# Autodesk Inventor assembly: CajaElectronica
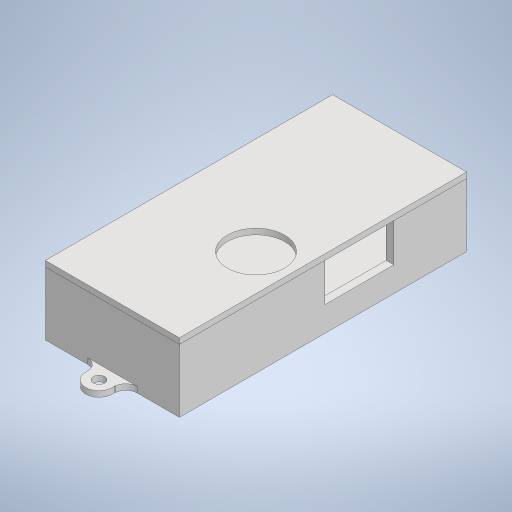
[picture p0: Inventor's stored thumbnail of the model, 512x512]
Saved by Autodesk Inventor 2024 (Build 280153000, 153)
## iProperties
Created: 2025-05-11
Part Number: CajaElectronica
Document SubType Name: Assembly
Designer: sergi
Author: sergi
## Documents named in this file (3)
- C:\Users\sergi\OneDrive\Escritorio\GitHub\08. VUmeter\Inventor\CajaElectronica.iam
- C:\Users\sergi\OneDrive\Escritorio\GitHub\08. VUmeter\Inventor\Caja.ipt
- C:\Users\sergi\OneDrive\Escritorio\GitHub\08. VUmeter\Inventor\Tapa.ipt
## Components (2 placed, 2 different names)
1. Caja:1 — Nivelación:1
2. Tapa:1 — Nivelación:1
## Relationships (1: Flush 1)
- Nivelación:1 [Flush]: Caja:1 ↔ Tapa:1
